# Autodesk Inventor assembly: 18x6-2F-CO-CCW v4
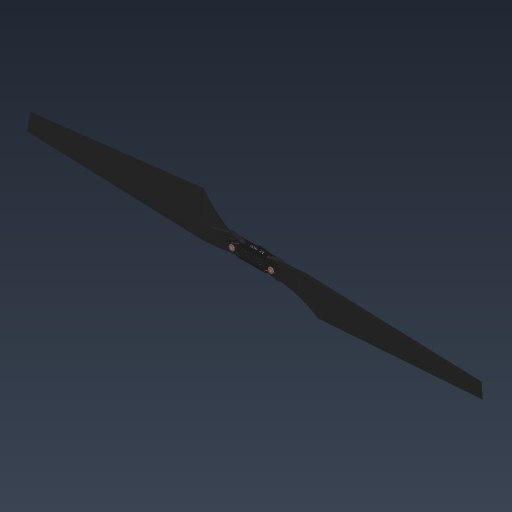
[picture p0: Inventor's stored thumbnail of the model, 512x512]
Saved by Autodesk Inventor 2024.1 (Build 281209000, 209)
## iProperties
RuleStatus: InUse
Created: 2023-12-07
Part Number: 18x6-2F-CO-CCW v4
Document SubType Name: Assembly
Designer: dzw04
Author: dzw04
## Documents named in this file (4)
- C:\Users\dzw04\Saxion\Mechatronica Lectoraat LMECH LED - Database ARG\Component_Database\SARAX\01. CAD\03. References\01. 3D_Files\Motor mount v12\18x6-2F-CO-CCW v4 v3.iam
- C:\Users\dzw04\Saxion\Mechatronica Lectoraat LMECH LED - Database ARG\Component_Database\SARAX\01. CAD\03. References\01. 3D_Files\Motor mount v12\T-Motor Folding Hub v2.iam
- C:\Users\dzw04\Saxion\Mechatronica Lectoraat LMECH LED - Database ARG\Component_Database\SARAX\01. CAD\03. References\01. 3D_Files\Motor mount v12\18x6-2F-CO CCW Blade v2.ipt
- C:\Users\dzw04\Saxion\Mechatronica Lectoraat LMECH LED - Database ARG\Component_Database\SARAX\01. CAD\03. References\01. 3D_Files\Motor mount v12\91290A113.ipt
## Components (5 placed, 3 different names)
1. T-Motor Folding Hub v2:1 [sub-assembly] — Mate:3, Mate:4, Angle:1, Angle:2
2. 18x6-2F-CO CCW Blade v2:1 — Mate:1, Mate:4, Angle:1
3. 18x6-2F-CO CCW Blade v2:2 — Mate:2, Mate:3, Angle:2
4. 91290A113:1 — Mate:1
5. 91290A113:2 — Mate:2
## Relationships (6: Mate 4, Angle 2)
- Mate:1: 18x6-2F-CO CCW Blade v2:1 ↔ 91290A113:1
- Mate:2: 18x6-2F-CO CCW Blade v2:2 ↔ 91290A113:2
- Mate:3: T-Motor Folding Hub v2:1 ↔ 18x6-2F-CO CCW Blade v2:2
- Mate:4: T-Motor Folding Hub v2:1 ↔ 18x6-2F-CO CCW Blade v2:1
- Angle:1 (0 deg): T-Motor Folding Hub v2:1 ↔ 18x6-2F-CO CCW Blade v2:1
- Angle:2 (0 deg): T-Motor Folding Hub v2:1 ↔ 18x6-2F-CO CCW Blade v2:2
